# Autodesk Inventor assembly: EnsamblajeSoporte
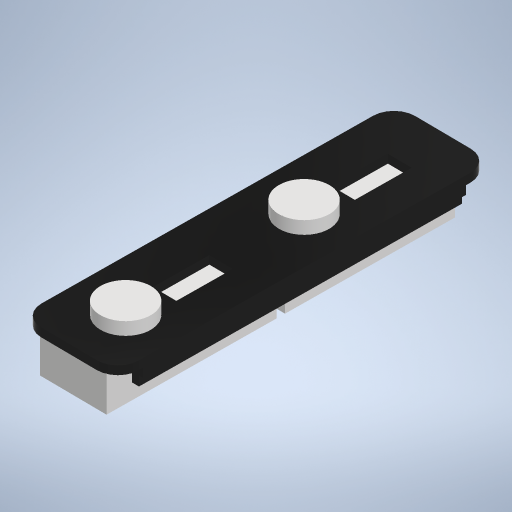
[picture p0: Inventor's stored thumbnail of the model, 512x512]
Saved by Autodesk Inventor 2024.1 (Build 281209000, 209)
## iProperties
Created: 2023-08-13
Part Number: EnsamblajeSoporte
Document SubType Name: Assembly
Designer: Det-Pc
Author: Det-Pc
## Documents named in this file (3)
- C:\Users\Det-Pc\Desktop\Tesis\Inventor\EnsamblajeSoporte.iam
- C:\Users\Det-Pc\Desktop\Tesis\Inventor\Soporte.ipt
- C:\Users\Det-Pc\Desktop\Tesis\Inventor\Cámara.ipt
## Components (3 placed, 2 different names)
1. Soporte:1 — Coincidencia:1, Coincidencia:2, Coincidencia:3, Coincidencia:4, Ángulo:1, Ángulo:2
2. Cámara:1 — Coincidencia:2, Coincidencia:4, Ángulo:1
3. Cámara:2 — Coincidencia:1, Coincidencia:3, Ángulo:2
## Relationships (6: Mate 4, Angle 2)
- Coincidencia:1 [Mate]: Soporte:1 ↔ Cámara:2
- Coincidencia:2 [Mate]: Soporte:1 ↔ Cámara:1
- Coincidencia:3 [Mate]: Soporte:1 ↔ Cámara:2
- Coincidencia:4 [Mate]: Soporte:1 ↔ Cámara:1
- Ángulo:1 [Angle] (90 deg): Soporte:1 ↔ Cámara:1
- Ángulo:2 [Angle] (90 deg): Soporte:1 ↔ Cámara:2
